# Autodesk Inventor assembly: slide assembly
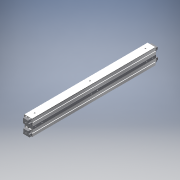
[picture p0: Inventor's stored thumbnail of the model, 180x180]
Saved by Autodesk Inventor 2019 (Build 230136000, 136)
## iProperties
Created: 2019-05-04
Part Number: slide assembly
Document SubType Name: Assembly
Designer: Delta
Author: Delta
## Documents named in this file (5)
- C:\Robotics\2019-20_CAD\offseason\random ideas\slides\slide assembly.iam
- C:\Robotics\2019-20_CAD\offseason\random ideas\slides\SAR330.iam
- C:\Robotics\2019-20_CAD\offseason\random ideas\slides\slide conector.ipt
- C:\Robotics\2019-20_CAD\offseason\random ideas\end peice for slides.ipt
- C:\Robotics\2019-20_CAD\offseason\random ideas\end peice for slides left.ipt
## Components (7 placed, 4 different names)
1. SAR330:1 [sub-assembly] — Mate:1, Mate:2, Mate:3, Mate:7, Mate:8, Flush:1, Mate:11, Flush:3, Mate:12
2. SAR330:2 [sub-assembly] — Mate:4, Mate:5, Mate:6, Mate:9, Mate:10, Flush:2, Mate:13, Flush:4, Mate:14
3. slide conector:1 — Mate:1, Mate:2, Mate:3, Mate:4, Mate:5, Mate:6
4. end peice for slides:1 — Mate:9, Mate:10, Flush:2
5. end peice for slides:2 — Mate:7, Mate:8, Flush:1
6. end peice for slides left:1 — Mate:11, Flush:3, Mate:12
7. end peice for slides left:2 — Mate:13, Flush:4, Mate:14
## Relationships (18: Mate 14, Flush 4)
- Mate:1: SAR330:1 ↔ slide conector:1
- Mate:2: SAR330:1 ↔ slide conector:1
- Mate:3: SAR330:1 ↔ slide conector:1
- Mate:4: SAR330:2 ↔ slide conector:1
- Mate:5: SAR330:2 ↔ slide conector:1
- Mate:6: SAR330:2 ↔ slide conector:1
- Mate:7: SAR330:1 ↔ end peice for slides:2
- Mate:8: SAR330:1 ↔ end peice for slides:2
- Flush:1: SAR330:1 ↔ end peice for slides:2
- Mate:9: SAR330:2 ↔ end peice for slides:1
- Mate:10: SAR330:2 ↔ end peice for slides:1
- Flush:2: SAR330:2 ↔ end peice for slides:1
- Mate:11: SAR330:1 ↔ end peice for slides left:1
- Flush:3: SAR330:1 ↔ end peice for slides left:1
- Mate:12: SAR330:1 ↔ end peice for slides left:1
- Mate:13: SAR330:2 ↔ end peice for slides left:2
- Flush:4: SAR330:2 ↔ end peice for slides left:2
- Mate:14: SAR330:2 ↔ end peice for slides left:2
